# Autodesk Inventor assembly: втулка+подшипники
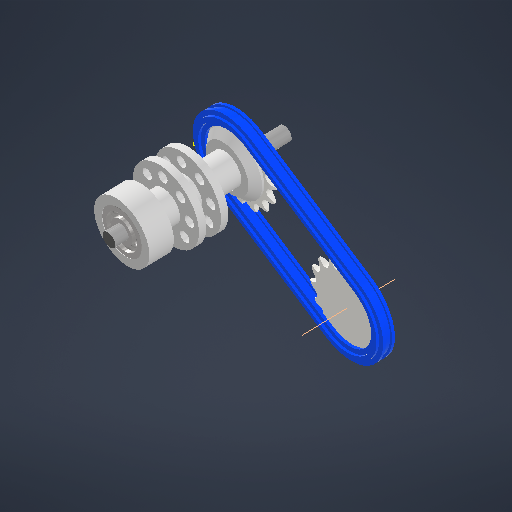
[picture p0: Inventor's stored thumbnail of the model, 512x512]
Saved by Autodesk Inventor 2025 (Build 290162000, 162)
## iProperties
Created: 2024-09-18
Part Number: втулка+подшипники
Document SubType Name: Assembly
Designer: GameHD
Sending System: Autodesk Inventor 2025
Preprocessor: ST-DEVELOPER v20
Author: Phantom
## Documents named in this file (5)
- C:\Users\GameHD\Desktop\Phantom 16950\втулка+подшипники нужная сборка.iam
- C:\Users\GameHD\Desktop\Phantom 16950\BS 290 SKF - SKF 626-RZ.ipt
- C:\Users\GameHD\Desktop\Phantom 16950\Деталь_64.ipt
- C:\Users\GameHD\Desktop\Phantom 16950\звезда и втулка.iam
- C:\Users\GameHD\Desktop\Phantom 16950\втулка для подш 2 часть.ipt
## Components (5 placed, 4 different names)
1. BS 290 SKF, с уплотнением с низким трением SKF 626-RZ:1 — Совмещение:1, Совмещение:4
2. BS 290 SKF, с уплотнением с низким трением SKF 626-RZ:2 — Совмещение:6, Совмещение:7
3. Деталь_64:1 — Совмещение:1, Совмещение:2, Совмещение:5, Совмещение:6
4. звезда и втулка:1 [sub-assembly] — Совмещение:2, Совмещение:3, Совмещение:7
5. втулка для подш 2 часть:1 — Совмещение:3, Совмещение:4, Совмещение:5
## Relationships (7: Mate 7)
- Совмещение:1 [Mate]: BS 290 SKF, с уплотнением с низким трением SKF 626-RZ:1 ↔ Деталь_64:1
- Совмещение:2 [Mate]: Деталь_64:1 ↔ звезда и втулка:1
- Совмещение:3 [Mate]: звезда и втулка:1 ↔ втулка для подш 2 часть:1
- Совмещение:4 [Mate]: BS 290 SKF, с уплотнением с низким трением SKF 626-RZ:1 ↔ втулка для подш 2 часть:1
- Совмещение:5 [Mate]: Деталь_64:1 ↔ втулка для подш 2 часть:1
- Совмещение:6 [Mate]: BS 290 SKF, с уплотнением с низким трением SKF 626-RZ:2 ↔ Деталь_64:1
- Совмещение:7 [Mate]: BS 290 SKF, с уплотнением с низким трением SKF 626-RZ:2 ↔ звезда и втулка:1
